# Autodesk Inventor assembly: 95658
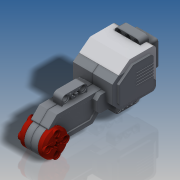
[picture p0: Inventor's stored thumbnail of the model, 180x180]
Saved by Autodesk Inventor 2016 SP2 (Build 200236200, 236)
## iProperties
Created: 2015-09-01
Part Number: 95658
Document SubType Name: Assembly
Designer: D. Kohfeld
Mass: 27.4433 g
Surface Area: 374.913 cm^2
Volume: 25.8899 cm^3
Density: 1.06 g/cm^3
Author: D. Kohfeld
## Documents named in this file (3)
- A:\LEGO Pieces\EV3\95658.iam
- A:\LEGO Pieces\EV3\99550c01.iam
- A:\LEGO Pieces\EV3\99617-Red.ipt
## Components (3 placed, 2 different names)
1. 99550c01:1 [sub-assembly] — Insert:1, Insert:2
2. 99617-Red:1 — Insert:2, Flush:1
3. 99617-Red:2 — Insert:1, Flush:1
## Relationships (3: Insert 2, Flush 1)
- Insert:1: 99550c01:1 ↔ 99617-Red:2
- Insert:2: 99550c01:1 ↔ 99617-Red:1
- Flush:1: 99617-Red:1 ↔ 99617-Red:2
